# Autodesk Inventor assembly: RGBLed
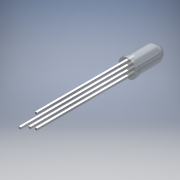
[picture p0: Inventor's stored thumbnail of the model, 180x180]
Saved by Autodesk Inventor 2019 (Build 230136000, 136)
## iProperties
Created: 2019-01-06
Part Number: RGBLed
Material: Generisch
Document SubType Name: Assembly
Designer: Jonas
Author: Jonas
## Documents named in this file (3)
- C:\Users\Jonas\Desktop\RGBCube\RGBCubev2\CAD\Led\RGBLed.iam
- C:\Users\Jonas\Desktop\RGBCube\RGBCubev2\CAD\Led\Head.ipt
- C:\Users\Jonas\Desktop\RGBCube\RGBCubev2\CAD\Led\Legs.ipt
## Components (2 placed, 2 different names)
1. Head:1 — Passend:1, Tangential:1, Passend:2
2. Legs:1 — Passend:1, Tangential:1, Passend:2
## Relationships (3: Mate 2, Tangent 1)
- Passend:1 [Mate] (-2 mm): Head:1 ↔ Legs:1
- Tangential:1 (-4.9 mm): Head:1 ↔ Legs:1
- Passend:2 [Mate] (-0.3 mm): Head:1 ↔ Legs:1
